# Autodesk Inventor assembly: redandblackBananaConnector
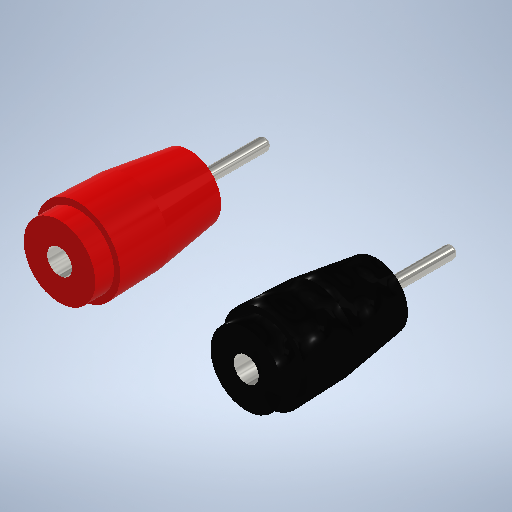
[picture p0: Inventor's stored thumbnail of the model, 512x512]
Saved by Autodesk Inventor 2025 (Build 290162000, 162)
## iProperties
Created: 2026-01-19
Part Number: redandblackBananaConnector
Document SubType Name: Assembly
Designer: tapen
Author: tapen
## Documents named in this file (3)
- C:\Users\tapen\OneDrive\Desktop\Chris Bidinosti\KVL+KCL\libs\3DModel\redandblackBananaConnector.iam
- C:\Users\tapen\OneDrive\Desktop\Chris Bidinosti\KVL+KCL\libs\3DModel\ipt\CT3149-0-Banana-Connector.ipt
- C:\Users\tapen\OneDrive\Desktop\Chris Bidinosti\KVL+KCL\libs\3DModel\ipt\CT3149-2-Banana-Connector.ipt
## Components (2 placed, 2 different names)
1. CT3149-2-Banana-Connector:1 — Mate:1, Flush:1, Mate:2, Mate:3
2. CT3149-0-Banana-Connector:1 — Flush:1, Mate:3
## Relationships (4: Mate 3, Flush 1)
- Mate:1: CT3149-2-Banana-Connector:1
- Flush:1: CT3149-2-Banana-Connector:1 ↔ CT3149-0-Banana-Connector:1
- Mate:2 (-15 mm): CT3149-2-Banana-Connector:1
- Mate:3 (30 mm): CT3149-2-Banana-Connector:1 ↔ CT3149-0-Banana-Connector:1
